# Autodesk Inventor assembly: 조립품4
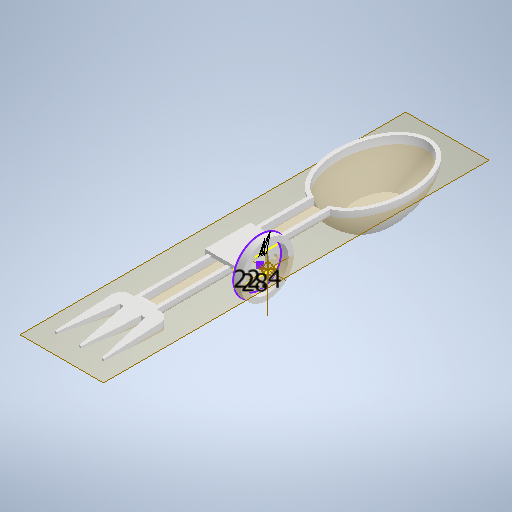
[picture p0: Inventor's stored thumbnail of the model, 512x512]
Saved by Autodesk Inventor 2026.1 (Build 301233020, 233B)
## iProperties
Created: 2025-09-20
Part Number: 조립품4
Document SubType Name: Assembly
Designer: wlgns
Author: wlgns
## Documents named in this file (3)
- C:\Users\wlgns\Desktop\Assistant Arm Project\ASSISTANT ARM MODEL\조립품4.iam
- C:\Users\wlgns\Desktop\Assistant Arm Project\ASSISTANT ARM MODEL\ASSISTANT ARM_origin\spoon.ipt
- C:\Users\wlgns\Desktop\Assistant Arm Project\ASSISTANT ARM MODEL\ASSISTANT ARM_origin\spoon2.ipt
## Components (2 placed, 2 different names)
1. spoon:1
2. spoon2:1 — 플러쉬:1, 메이트:1, 메이트:2
## Relationships (3: Mate 2, Flush 1)
- 플러쉬:1 [Flush]: spoon2:1
- 메이트:1 [Mate]: spoon2:1
- 메이트:2 [Mate]: spoon2:1
